# Autodesk Inventor assembly: Display
(part 2 of 2)
263. Open CASCADE STEP translator 7.5 263
264. Open CASCADE STEP translator 7.5 264
265. Open CASCADE STEP translator 7.5 265
266. Open CASCADE STEP translator 7.5 266
267. Open CASCADE STEP translator 7.5 267
268. Open CASCADE STEP translator 7.5 268
269. Open CASCADE STEP translator 7.5 269
270. Open CASCADE STEP translator 7.5 270
271. Open CASCADE STEP translator 7.5 271
272. Open CASCADE STEP translator 7.5 272
273. Open CASCADE STEP translator 7.5 273
274. Open CASCADE STEP translator 7.5 274
275. Open CASCADE STEP translator 7.5 275
276. Open CASCADE STEP translator 7.5 276
277. Open CASCADE STEP translator 7.5 277
278. Open CASCADE STEP translator 7.5 278
279. Open CASCADE STEP translator 7.5 279
280. Open CASCADE STEP translator 7.5 280
281. Open CASCADE STEP translator 7.5 281
282. Open CASCADE STEP translator 7.5 282
283. Open CASCADE STEP translator 7.5 283
284. Open CASCADE STEP translator 7.5 284
285. Open CASCADE STEP translator 7.5 285
286. Open CASCADE STEP translator 7.5 286
287. Open CASCADE STEP translator 7.5 287
288. Open CASCADE STEP translator 7.5 288
289. Open CASCADE STEP translator 7.5 289
290. Open CASCADE STEP translator 7.5 290
291. Open CASCADE STEP translator 7.5 291
292. Open CASCADE STEP translator 7.5 292
293. Open CASCADE STEP translator 7.5 293
294. Open CASCADE STEP translator 7.5 294
295. Open CASCADE STEP translator 7.5 295
296. Open CASCADE STEP translator 7.5 296
297. Open CASCADE STEP translator 7.5 297
298. Open CASCADE STEP translator 7.5 298
299. Open CASCADE STEP translator 7.5 299
300. Open CASCADE STEP translator 7.5 300
301. Open CASCADE STEP translator 7.5 301
302. Open CASCADE STEP translator 7.5 302
303. Open CASCADE STEP translator 7.5 303
304. Open CASCADE STEP translator 7.5 304
305. Open CASCADE STEP translator 7.5 305
306. Open CASCADE STEP translator 7.5 306
307. Open CASCADE STEP translator 7.5 307
308. Open CASCADE STEP translator 7.5 308
309. Open CASCADE STEP translator 7.5 309
310. Open CASCADE STEP translator 7.5 310
311. Open CASCADE STEP translator 7.5 311
312. Open CASCADE STEP translator 7.5 312
313. Open CASCADE STEP translator 7.5 313
314. Open CASCADE STEP translator 7.5 314
315. Open CASCADE STEP translator 7.5 315
316. Open CASCADE STEP translator 7.5 316
